# Autodesk Inventor assembly: 211-02
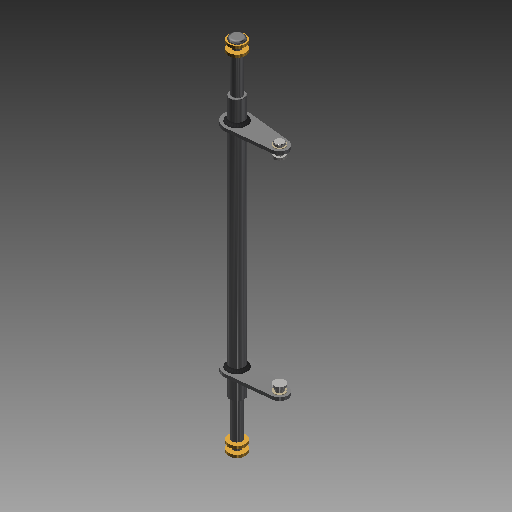
[picture p0: Inventor's stored thumbnail of the model, 512x512]
Saved by Autodesk Inventor 2019 (Build 230136000, 136)
## iProperties
Company: Autodesk Inc.
Created: 2007-12-25
Part Number: 211-02
Document SubType Name: Assembly
Designer: Autodesk Inc.
Mass: 639.761 g
Surface Area: 331.874 cm^2
Volume: 81.6607 cm^3
Density: 7.83438 g/cm^3
Description: FRONT PIVOT LINK ASSEMBLY
Component Category: Lower Component
Author: Inventor
## Documents named in this file (5)
- C:\TEMP\Car Seat\Workspace\Front Pivot Links.iam
- C:\TEMP\Car Seat\Workspace\Front Pivot Weldment.iam
- C:\TEMP\Car Seat\Workspace\Pivot Pin C.ipt
- C:\TEMP\Car Seat\Workspace\Bushing 2.ipt
- C:\TEMP\Car Seat\Workspace\Brass Spacer.ipt
## Components (9 placed, 4 different names)
1. Front Pivot Weldment:1 [sub-assembly] — Insert:1, Insert:2, Angle:1, Angle:2, Insert:5, Insert:7
2. Bushing 2:1 — Insert:1, Angle:1, Insert:3
3. Bushing 2:2 — Insert:2, Angle:2, Insert:4
4. Pivot Pin C:1 — Insert:3
5. Pivot Pin C:2 — Insert:4
6. Brass Spacer:1 — Insert:5, Insert:6
7. Brass Spacer:2 — Insert:6
8. Brass Spacer:3 — Insert:8
9. Brass Spacer:4 — Insert:7, Insert:8
## Relationships (10: Insert 8, Angle 2)
- Insert:1: Front Pivot Weldment:1 ↔ Bushing 2:1
- Insert:2: Front Pivot Weldment:1 ↔ Bushing 2:2
- Angle:1 (0 deg): Front Pivot Weldment:1 ↔ Bushing 2:1
- Angle:2 (180 deg): Front Pivot Weldment:1 ↔ Bushing 2:2
- Insert:3: Bushing 2:1 ↔ Pivot Pin C:1
- Insert:4: Bushing 2:2 ↔ Pivot Pin C:2
- Insert:5: Front Pivot Weldment:1 ↔ Brass Spacer:1
- Insert:6 (5.5 mm): Brass Spacer:1 ↔ Brass Spacer:2
- Insert:7: Front Pivot Weldment:1 ↔ Brass Spacer:4
- Insert:8 (5.5 mm): Brass Spacer:3 ↔ Brass Spacer:4
